# Autodesk Inventor assembly: case_with_gopro_mount
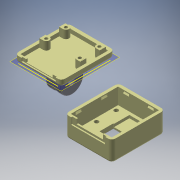
[picture p0: Inventor's stored thumbnail of the model, 180x180]
Saved by Autodesk Inventor 2019 (Build 230136000, 136)
## iProperties
Created: 2019-02-05
Part Number: case_with_gopro_mount
Document SubType Name: Assembly
Designer: jmc
Author: jmc
## Documents named in this file (4)
- C:\Users\l0086\Desktop\Models\3party\raspberry case hdmi\case_with_gopro_mount.iam
- C:\Users\l0086\Desktop\Models\3party\Gopro\gopro_male_connector.ipt
- C:\Users\l0086\Desktop\Models\3party\raspberry case hdmi\hdmicase_bottom_clean.ipt
- C:\Users\l0086\Desktop\Models\3party\raspberry case hdmi\hdmicase_top_clean.ipt
## Components (3 placed, 3 different names)
1. hdmicase_bottom_clean:1
2. hdmicase_top_clean:1 — Rigid:1
3. gopro_male_connector:1 — Rigid:1
## Relationships (1: WeldJoint 1)
- Rigid:1 [WeldJoint]: hdmicase_top_clean:1 ↔ gopro_male_connector:1
